# Autodesk Inventor assembly: tensioner2
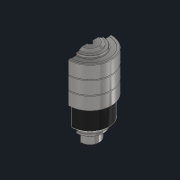
[picture p0: Inventor's stored thumbnail of the model, 180x180]
Saved by Autodesk Inventor 2022 (Build 260153000, 153)
## iProperties
Created: 2021-07-18
Part Number: tensioner2
Document SubType Name: Assembly
Designer: yuta0
Mass: 26.9565 g
Surface Area: 38.6954 cm^2
Volume: 3.73485 cm^3
Density: 7.21757 g/cm^3
Author: yuta0
## Documents named in this file (7)
- C:\Users\yuta0\Documents\GitHub\catchrobo_hardware\assy-robot\tensioner2.iam
- C:\Users\yuta0\Documents\GitHub\catchrobo_hardware\assy-robot\B688ZZ.ipt
- C:\Users\yuta0\Documents\GitHub\catchrobo_hardware\assy-robot\WSJ-STN-M4.ipt
- C:\Users\yuta0\Documents\GitHub\catchrobo_hardware\assy-robot\CBSTSR4-6.ipt
- C:\Users\yuta0\Documents\GitHub\catchrobo_hardware\assy-robot\base40.ipt
- C:\Users\yuta0\Documents\GitHub\catchrobo_hardware\assy-robot\CB4-10.ipt
- C:\Users\yuta0\Documents\GitHub\catchrobo_hardware\assy-robot\SFHRW8-20-M4-N4_s.ipt
## Components (9 placed, 6 different names)
1. CB4-10:1 — メイト:20, メイト:21
2. WSJ-STN-M4:1 — メイト:15, メイト:27, メイト:28, メイト:30
3. WSJ-STN-M4:2 — メイト:18, メイト:19, メイト:20, メイト:21
4. CBSTSR4-6:1 — メイト:15, メイト:30
5. base40:1 — メイト:18, メイト:19, メイト:22, メイト:24, メイト:26
6. SFHRW8-20-M4-N4_s:1 — メイト:24, メイト:25, メイト:26, メイト:29
7. B688ZZ:1 — メイト:22, メイト:29
8. B688ZZ:2 — メイト:25
9. B688ZZ:3 — メイト:27, メイト:28
## Component patterns: (3 elements, first: B688ZZ:1)
## Relationships (13: Mate 13)
- メイト:15 [Mate]: WSJ-STN-M4:1 ↔ CBSTSR4-6:1
- メイト:18 [Mate] (2 mm): WSJ-STN-M4:2 ↔ base40:1
- メイト:19 [Mate]: WSJ-STN-M4:2 ↔ base40:1
- メイト:20 [Mate]: CB4-10:1 ↔ WSJ-STN-M4:2
- メイト:21 [Mate]: CB4-10:1 ↔ WSJ-STN-M4:2
- メイト:22 [Mate]: base40:1 ↔ B688ZZ:1
- メイト:24 [Mate]: base40:1 ↔ SFHRW8-20-M4-N4_s:1
- メイト:25 [Mate]: SFHRW8-20-M4-N4_s:1 ↔ B688ZZ:2
- メイト:26 [Mate]: base40:1 ↔ SFHRW8-20-M4-N4_s:1
- メイト:27 [Mate]: WSJ-STN-M4:1 ↔ B688ZZ:3
- メイト:28 [Mate]: WSJ-STN-M4:1 ↔ B688ZZ:3
- メイト:29 [Mate]: SFHRW8-20-M4-N4_s:1 ↔ B688ZZ:1
- メイト:30 [Mate]: WSJ-STN-M4:1 ↔ CBSTSR4-6:1
